# Autodesk Inventor assembly: 試作1
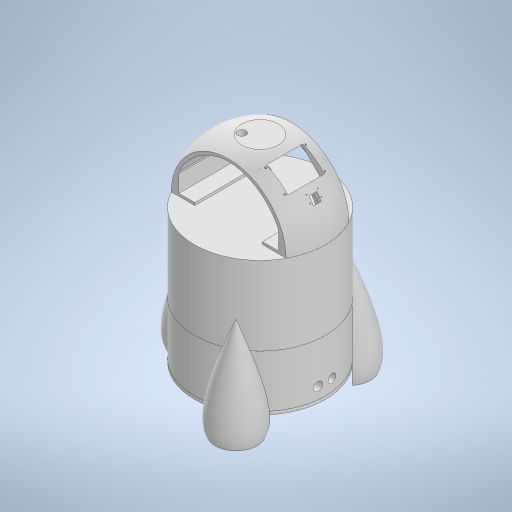
[picture p0: Inventor's stored thumbnail of the model, 512x512]
Saved by Autodesk Inventor 2023 (Build 270158000, 158)
## iProperties
Created: 2022-11-18
Part Number: 試作1
Document SubType Name: Assembly
Designer: 野口　裕太
Author: 野口　裕太
## Documents named in this file (7)
- D:\ロボ創\試作1.iam
- D:\ロボ創\底板 (2).ipt
- D:\ロボ創\newbody6.ipt
- D:\ロボ創\newbody5.ipt
- D:\ロボ創\newleg.ipt
- D:\ロボ創\dummy1.ipt
- D:\ロボ創\newhead.ipt
## Components (9 placed, 6 different names)
1. 底板 (2):1 — メイト:1, メイト:2, メイト:3, メイト:4, メイト:5, メイト:6, メイト:8, メイト:9, メイト:10
2. newbody6:1 — メイト:1, メイト:2, メイト:3, メイト:7, メイト:12, メイト:13
3. newbody5:1 — メイト:8, メイト:9, メイト:10, メイト:11, メイト:18
4. newbody5:2 — メイト:4, メイト:5, メイト:6, メイト:7, メイト:14, メイト:15, メイト:16, メイト:17
5. newleg:1 — メイト:13, メイト:14
6. newleg:2 — メイト:11, メイト:12
7. newleg:3 — メイト:15, メイト:16
8. dummy1:1 — メイト:17, メイト:18, メイト:19, メイト:20
9. newhead:1 — メイト:19, メイト:20
## Relationships (20: Mate 20)
- メイト:1 [Mate]: 底板 (2):1 ↔ newbody6:1
- メイト:2 [Mate]: 底板 (2):1 ↔ newbody6:1
- メイト:3 [Mate]: 底板 (2):1 ↔ newbody6:1
- メイト:4 [Mate]: 底板 (2):1 ↔ newbody5:2
- メイト:5 [Mate]: 底板 (2):1 ↔ newbody5:2
- メイト:6 [Mate]: 底板 (2):1 ↔ newbody5:2
- メイト:7 [Mate]: newbody6:1 ↔ newbody5:2
- メイト:8 [Mate]: 底板 (2):1 ↔ newbody5:1
- メイト:9 [Mate]: 底板 (2):1 ↔ newbody5:1
- メイト:10 [Mate]: 底板 (2):1 ↔ newbody5:1
- メイト:11 [Mate]: newbody5:1 ↔ newleg:2
- メイト:12 [Mate]: newbody6:1 ↔ newleg:2
- メイト:13 [Mate]: newbody6:1 ↔ newleg:1
- メイト:14 [Mate]: newbody5:2 ↔ newleg:1
- メイト:15 [Mate]: newbody5:2 ↔ newleg:3
- メイト:16 [Mate]: newbody5:2 ↔ newleg:3
- メイト:17 [Mate]: newbody5:2 ↔ dummy1:1
- メイト:18 [Mate]: newbody5:1 ↔ dummy1:1
- メイト:19 [Mate]: dummy1:1 ↔ newhead:1
- メイト:20 [Mate]: dummy1:1 ↔ newhead:1
